# Autodesk Inventor assembly: Assembled_gameMechanicstest
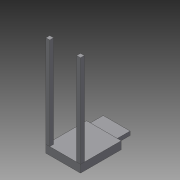
[picture p0: Inventor's stored thumbnail of the model, 180x180]
Saved by Autodesk Inventor 2015 (Build 190159000, 159)
## iProperties
Created: 2015-01-15
Part Number: Assembled_gameMechanicstest
Document SubType Name: Assembly
Designer: Tucker
Author: Tucker
## Documents named in this file (4)
- C:\Users\Tucker\Documents\GitHub\frc2015\CAD\Assembled_gameMechanicstest.iam
- C:\Users\Tucker\Documents\GitHub\frc2015\CAD\chasse.ipt
- C:\Users\Tucker\Documents\GitHub\frc2015\CAD\pole.ipt
- C:\Users\Tucker\Documents\GitHub\frc2015\CAD\box_forklift.ipt
## Components (4 placed, 3 different names)
1. chasse:1 — Mate:1, Flush:1, Flush:2, Mate:2, Flush:3, Flush:4, Mate:3
2. pole:1 — Mate:1, Flush:1, Flush:2
3. pole:2 — Mate:2, Flush:3, Flush:4
4. box_forklift:1 — Mate:3
## Relationships (7: Flush 4, Mate 3)
- Mate:1: chasse:1 ↔ pole:1
- Flush:1: chasse:1 ↔ pole:1
- Flush:2: chasse:1 ↔ pole:1
- Mate:2: chasse:1 ↔ pole:2
- Flush:3: chasse:1 ↔ pole:2
- Flush:4: chasse:1 ↔ pole:2
- Mate:3: chasse:1 ↔ box_forklift:1
